# Autodesk Inventor assembly: Rocket Assembly
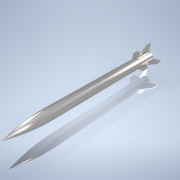
[picture p0: Inventor's stored thumbnail of the model, 180x180]
Saved by Autodesk Inventor 2022 (Build 260153000, 153)
## iProperties
Created: 2021-10-30
Part Number: Rocket Assembly
Document SubType Name: Assembly
Designer: Ryan
Author: Ryan
## Documents named in this file (7)
- C:\GitHub\ENAE100-Project\Rocket Assembly.iam
- C:\GitHub\ENAE100-Project\Nose Cone.ipt
- C:\GitHub\ENAE100-Project\Centering Ring.ipt
- C:\GitHub\ENAE100-Project\Motor Mount.ipt
- C:\GitHub\ENAE100-Project\Motor.ipt
- C:\GitHub\ENAE100-Project\Fin.ipt
- C:\GitHub\ENAE100-Project\Body Tube.ipt
## Components (10 placed, 6 different names)
1. Nose Cone:1 — Rigid:1
2. Centering Ring:1 — Rigid:3
3. Centering Ring:2 — Rigid:2
4. Motor Mount:1 — Rigid:4
5. Motor:1 — Rotational:1
6. Fin:1 — Rigid:6
7. Fin:2 — Rigid:7
8. Fin:3 — Rigid:8
9. Fin:4 — Rigid:5
10. Body Tube:1 — Rigid:1, Rigid:2, Rigid:3, Rigid:4, Rotational:1, Rigid:5, Rigid:6, Rigid:7, Rigid:8
## Relationships (9: WeldJoint 8, RevoluteJoint 1)
- Rigid:1 [WeldJoint]: Nose Cone:1 ↔ Body Tube:1
- Rigid:2 [WeldJoint] (-114.3 mm): Centering Ring:2 ↔ Body Tube:1
- Rigid:3 [WeldJoint] (-12.7 mm): Centering Ring:1 ↔ Body Tube:1
- Rigid:4 [WeldJoint]: Motor Mount:1 ↔ Body Tube:1
- Rotational:1 [RevoluteJoint]: Motor:1 ↔ Body Tube:1
- Rigid:5 [WeldJoint]: Fin:4 ↔ Body Tube:1
- Rigid:6 [WeldJoint]: Fin:1 ↔ Body Tube:1
- Rigid:7 [WeldJoint]: Fin:2 ↔ Body Tube:1
- Rigid:8 [WeldJoint]: Fin:3 ↔ Body Tube:1
